# Autodesk Inventor assembly: Blue Alliance Bucket
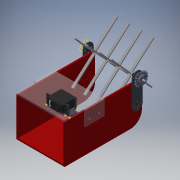
[picture p0: Inventor's stored thumbnail of the model, 180x180]
Saved by Autodesk Inventor 2016 (Build 200138000, 138)
## iProperties
Created: 2015-12-16
Part Number: Blue Alliance Bucket
Document SubType Name: Assembly
Designer: TimB
Author: TimB
## Documents named in this file (12)
- C:\Users\tbloo\Documents\GitHub\phi_robotics\3d-models\FTC_Tetrix_KOP_Block_Party\Tim Bloot Designs\JAr JaR Bot\Red Alliance Bucket.iam
- C:\Users\tbloo\Documents\GitHub\phi_robotics\3d-models\FTC_Tetrix_KOP_Block_Party\Tetrix_Kit_FTC\Autodesk Inventor Files\tetrix_servo_mount.ipt
- C:\Users\tbloo\Documents\GitHub\phi_robotics\3d-models\FTC_Tetrix_KOP_Block_Party\Tetrix_Kit_FTC\Autodesk Inventor Files\tetrix_739061_2012.ipt
- C:\Users\tbloo\Documents\GitHub\phi_robotics\3d-models\FTC_Tetrix_KOP_Block_Party\Tim Bloot Designs\JAr JaR Bot\Bucket -  Top.ipt
- C:\Users\tbloo\Documents\GitHub\phi_robotics\3d-models\FTC_Tetrix_KOP_Block_Party\Tetrix_Kit_FTC\Autodesk Inventor Files\tetrix_servo_body.ipt
- C:\Users\tbloo\Documents\GitHub\phi_robotics\3d-models\FTC_Tetrix_KOP_Block_Party\Tetrix_Kit_FTC\Autodesk Inventor Files\tetrix_739092_2012.iam
- C:\Users\tbloo\Documents\GitHub\phi_robotics\3d-models\FTC_Tetrix_KOP_Block_Party\Tetrix_Kit_FTC\Autodesk Inventor Files\tetrix_bushing.ipt
- C:\Users\tbloo\Documents\GitHub\phi_robotics\3d-models\FTC_Tetrix_KOP_Block_Party\Tim Bloot Designs\JAr JaR Bot\Bucket - 4 Rake.iam
- C:\Users\tbloo\Documents\GitHub\phi_robotics\3d-models\FTC_Tetrix_KOP_Block_Party\Tim Bloot Designs\JAr JaR Bot\Bucket - Axle.ipt
- C:\Users\tbloo\Documents\GitHub\phi_robotics\3d-models\FTC_Tetrix_KOP_Block_Party\Tetrix_Kit_FTC\Autodesk Inventor Files\tetrix_axle_lock.iam
- C:\Users\tbloo\Documents\GitHub\phi_robotics\3d-models\FTC_Tetrix_KOP_Block_Party\Tetrix_Kit_FTC\Autodesk Inventor Files\tetrix_chain_gear-16t.ipt
- C:\Users\tbloo\Documents\GitHub\phi_robotics\3d-models\FTC_Tetrix_KOP_Block_Party\Tim Bloot Designs\JAr JaR Bot\Bucket - RedA.ipt
## Components (13 placed, 11 different names)
1. tetrix_739061_2012:1 — Rotational:3, Rigid:13
2. tetrix_739061_2012:2 — Rotational:4, Rigid:14
3. Bucket -  Top:1 — Rigid:9, Rigid:12
4. tetrix_739092_2012:2 [sub-assembly] — Rotational:5, Rigid:6
5. tetrix_bushing:1 — Rotational:3
6. Bucket - 4 Rake:1 [sub-assembly] — Rigid:7
7. tetrix_bushing:2 — Rotational:4, Rotational:5
8. Bucket - Axle:1 — Rigid:6, Rigid:7, Rigid:11
9. tetrix_servo_mount:1 — Rigid:8, Rigid:9
10. tetrix_servo_body:2 — Rigid:8
11. tetrix_axle_lock:1 [sub-assembly] — Rigid:11
12. tetrix_chain_gear-16t:1
13. Bucket - RedA:1 — Rigid:12, Rigid:13, Rigid:14
## Relationships (12: WeldJoint 9, RevoluteJoint 3)
- Rotational:3 [RevoluteJoint]: tetrix_739061_2012:1 ↔ tetrix_bushing:1
- Rotational:4 [RevoluteJoint]: tetrix_739061_2012:2 ↔ tetrix_bushing:2
- Rotational:5 [RevoluteJoint]: tetrix_739092_2012:2 ↔ tetrix_bushing:2
- Rigid:6 [WeldJoint]: tetrix_739092_2012:2 ↔ Bucket - Axle:1
- Rigid:7 [WeldJoint] (-10 mm): Bucket - 4 Rake:1 ↔ Bucket - Axle:1
- Rigid:8 [WeldJoint]: tetrix_servo_mount:1 ↔ tetrix_servo_body:2
- Rigid:9 [WeldJoint]: Bucket -  Top:1 ↔ tetrix_servo_mount:1
- [WeldJoint]: tetrix_axle_lock:1 ↔ tetrix_chain_gear-16t:1
- Rigid:11 [WeldJoint] (-19.6 mm): Bucket - Axle:1 ↔ tetrix_axle_lock:1
- Rigid:12 [WeldJoint]: Bucket -  Top:1 ↔ Bucket - RedA:1
- Rigid:13 [WeldJoint]: tetrix_739061_2012:1 ↔ Bucket - RedA:1
- Rigid:14 [WeldJoint]: tetrix_739061_2012:2 ↔ Bucket - RedA:1
## Named parameters: d30_d15 = 0 mm
